# Autodesk Inventor assembly: wahacz_srodkowy_zlozenie_kopia
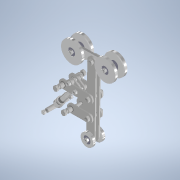
[picture p0: Inventor's stored thumbnail of the model, 180x180]
Saved by Autodesk Inventor 2020.3 (Build 243373000, 373)
## iProperties
Created: 2021-10-24
Part Number: wahacz_srodkowy_zlozenie_kopia
Document SubType Name: Assembly
Designer: patry
Author: patry
## Documents named in this file (28)
- C:\Users\patry\Desktop\Semestr 7\Inzynierka\Projekt inventor\Ariadna_inzynierka\Workspaces\Obszar roboczy\Obszar roboczy\Naped\Zawieszenie_v3\wahacz_srodkowy_zlozenie_kopia.iam
- C:\Users\patry\Desktop\Semestr 7\Inzynierka\Projekt inventor\Ariadna_inzynierka\Workspaces\Obszar roboczy\Obszar roboczy\Naped\Zawieszenie_v3\glowny_wahacz.ipt
- C:\Users\patry\Desktop\Semestr 7\Inzynierka\Projekt inventor\Ariadna_inzynierka\Workspaces\Obszar roboczy\Obszar roboczy\Naped\Zawieszenie_v3\ramie_1_wahacza.ipt
- C:\Users\patry\Desktop\Semestr 7\Inzynierka\Projekt inventor\Ariadna_inzynierka\Workspaces\Obszar roboczy\Obszar roboczy\Naped\Zawieszenie_v3\ramie_2_wahacza.ipt
- C:\Users\patry\Desktop\Semestr 7\Inzynierka\Projekt inventor\Ariadna_inzynierka\Workspaces\Obszar roboczy\Obszar roboczy\Naped\Zawieszenie_v3\tuleja_TUF106040.ipt
- C:\Users\patry\Desktop\Semestr 7\Inzynierka\Projekt inventor\Ariadna_inzynierka\Workspaces\Obszar roboczy\Obszar roboczy\Naped\Zawieszenie_v3\komplet_kol_V4.iam
- C:\Users\patry\Desktop\Semestr 7\Inzynierka\Projekt inventor\Ariadna_inzynierka\Workspaces\Obszar roboczy\Obszar roboczy\Naped\Sruby\M6_nut_5mm.ipt
- C:\Users\patry\Desktop\Semestr 7\Inzynierka\Projekt inventor\Ariadna_inzynierka\Workspaces\Obszar roboczy\Obszar roboczy\Naped\Amortyzator\Korpus.ipt
- C:\Users\patry\Desktop\Semestr 7\Inzynierka\Projekt inventor\Ariadna_inzynierka\Workspaces\Obszar roboczy\Obszar roboczy\Naped\Amortyzator\Tlok.ipt
- C:\Users\patry\Desktop\Semestr 7\Inzynierka\Projekt inventor\Ariadna_inzynierka\Workspaces\Obszar roboczy\Obszar roboczy\Naped\Amortyzator\Nakretka.ipt
- C:\Users\patry\Desktop\Semestr 7\Inzynierka\Projekt inventor\Ariadna_inzynierka\Workspaces\Obszar roboczy\Obszar roboczy\Naped\Sruby\M5_nut_5mm.ipt
- C:\Users\patry\Desktop\Semestr 7\Inzynierka\Projekt inventor\Ariadna_inzynierka\Workspaces\Obszar roboczy\Obszar roboczy\Naped\Sruby\M6_25_shaft.ipt
- C:\Users\patry\Desktop\Semestr 7\Inzynierka\Projekt inventor\Ariadna_inzynierka\Workspaces\Obszar roboczy\Obszar roboczy\Naped\Sruby\M5_70_shaft.ipt
- C:\Users\patry\Desktop\Semestr 7\Inzynierka\Projekt inventor\Ariadna_inzynierka\Workspaces\Obszar roboczy\Obszar roboczy\Naped\Sruby\M3_16_shaft.ipt
- C:\Users\patry\Desktop\Semestr 7\Inzynierka\Projekt inventor\Ariadna_inzynierka\Workspaces\Obszar roboczy\Obszar roboczy\Naped\Sruby\M3_nut_2,5mm.ipt
- C:\Users\patry\Desktop\Semestr 7\Inzynierka\Projekt inventor\Ariadna_inzynierka\Workspaces\Obszar roboczy\Obszar roboczy\Naped\Zawieszenie_v3\wspornik_amortyzatora.ipt
- C:\Users\patry\Desktop\Semestr 7\Inzynierka\Projekt inventor\Ariadna_inzynierka\Workspaces\Obszar roboczy\Obszar roboczy\Naped\Sruby\M6_40_shaft.ipt
- C:\Users\patry\Desktop\Semestr 7\Inzynierka\Projekt inventor\Ariadna_inzynierka\Workspaces\Obszar roboczy\Obszar roboczy\Naped\Sruby\tuleja_M6_M10_7.ipt
- C:\Users\patry\Desktop\Semestr 7\Inzynierka\Projekt inventor\Ariadna_inzynierka\Workspaces\Obszar roboczy\Obszar roboczy\Naped\Sruby\M6_1,25_pad.ipt
- C:\Users\patry\Desktop\Semestr 7\Inzynierka\Projekt inventor\Ariadna_inzynierka\Workspaces\Obszar roboczy\Obszar roboczy\Naped\Sruby\M6_70_shaft.ipt
- C:\Users\patry\Desktop\Semestr 7\Inzynierka\Projekt inventor\Ariadna_inzynierka\Workspaces\Obszar roboczy\Obszar roboczy\Naped\Sruby\M5_40_shaft.ipt
- M5_shaft.ipt
- C:\Users\patry\Desktop\Semestr 7\Inzynierka\Projekt inventor\Ariadna_inzynierka\Workspaces\Obszar roboczy\Obszar roboczy\Naped\Sruby\tuleja_M5_M9_20.ipt
- C:\Users\patry\Desktop\Semestr 7\Inzynierka\Projekt inventor\Ariadna_inzynierka\Workspaces\Obszar roboczy\Obszar roboczy\Naped\Sruby\tuleja_M5_M9_25.ipt
- C:\Users\patry\Desktop\Semestr 7\Inzynierka\Projekt inventor\Ariadna_inzynierka\Workspaces\Obszar roboczy\Obszar roboczy\Naped\Sruby\tuleja_M5_M9_4,5.ipt
- C:\Users\patry\Desktop\Semestr 7\Inzynierka\Projekt inventor\Ariadna_inzynierka\Workspaces\Obszar roboczy\Obszar roboczy\Naped\Kola\holder_wheel_pair.iam
- C:\Users\patry\Desktop\Semestr 7\Inzynierka\Projekt inventor\Ariadna_inzynierka\Workspaces\Obszar roboczy\Obszar roboczy\Naped\Sruby\tuleja_M6_M10_8,5.ipt
- C:\Users\patry\Desktop\Semestr 7\Inzynierka\Projekt inventor\Ariadna_inzynierka\Workspaces\Obszar roboczy\Obszar roboczy\Naped\Sruby\tuleja_M6_M10_13,5.ipt
## Components (68 placed, 26 different names)
1. glowny_wahacz:1 — Zestawiające:9, Zestawiające:12, Zestawiające:23, Zestawiające:35, Zestawiające:79, Zestawiające:106, Zestawiające:107, Zestawiające:122, Zestawiające:128, Zestawiające:136
2. ramie_1_wahacza:1 — Zestawiające:7, Zestawiające:8, Kątowe:4, Zestawiające:108, Zestawiające:109, Zestawiające:110, Równoległe:6, Zestawiające:114, Zestawiające:158, Równoległe:11, Zestawiające:159, Równoległe:12, Zestawiające:161, Zestawiające:163, Zestawiające:175, Zestawiające:179, Zestawiające:191, Zestawiające:192
3. ramie_2_wahacza:1 — Zestawiające:1, Zestawiające:2, Kątowe:1, Zestawiające:118, Zestawiające:185, Zestawiające:186
4. tuleja_TUF106040:1 — Zestawiające:1, Zestawiające:2, Kątowe:1, Zestawiające:23, Zestawiające:93
5. tuleja_TUF106040:2 — Zestawiające:184, Zestawiające:185, Zestawiające:186, Zestawiające:196
6. tuleja_TUF106040:3 — Zestawiające:190, Zestawiające:191, Zestawiające:192, Zestawiające:200
7. tuleja_TUF106040:4 — Zestawiające:7, Zestawiające:8, Kątowe:4, Zestawiające:104, Zestawiające:105, Zestawiające:111, Zestawiające:132
8. komplet_kol_V4:1 [sub-assembly] — Zestawiające:9, Zestawiające:10, Zestawiające:11, Zestawiające:12, Równoległe:13
9. glowny_wahacz:2 — Zestawiające:10, Zestawiające:11, Zestawiające:29, Zestawiające:79, Zestawiające:80, Równoległe:3, Zestawiające:82, Zestawiające:92, Zestawiające:104, Zestawiające:105, Zestawiające:124, Zestawiające:180
10. tuleja_TUF106040:5 — Zestawiające:187, Zestawiające:188, Zestawiające:189, Zestawiające:198
11. tuleja_TUF106040:6 — Zestawiające:88, Zestawiające:90, Zestawiające:106, Zestawiające:107
12. ramie_2_wahacza:2 — Równoległe:7, Zestawiające:120, Zestawiające:182, Zestawiające:183
13. tuleja_TUF106040:7 — Zestawiające:29, Zestawiające:92, Zestawiające:93, Zestawiające:112, Zestawiające:140
14. tuleja_TUF106040:8 — Zestawiające:181, Zestawiające:182, Zestawiające:183, Zestawiające:194
15. M6_nut_5mm:1 — Zestawiające:35
16. M6_nut_5mm:2 — Zestawiające:113, Zestawiające:114
17. Korpus:1 — Walcowe:1, Zestawiające:83, Równoległe:4, Zestawiające:87, Zestawiające:169, Zestawiające:171
18. Tlok:1 — Walcowe:1, Zestawiające:102, Zestawiające:103
19. Nakretka:1
20. M5_nut_5mm:1 — Zestawiające:84, Zestawiające:86, Zestawiające:87, Równoległe:9, Równoległe:10
21. M6_25_shaft:1 — Zestawiające:80, Równoległe:3, Zestawiające:81
22. M6_nut_5mm:10 — Zestawiające:81, Zestawiające:82
23. M5_70_shaft:1 — Zestawiające:83, Równoległe:4, Zestawiające:84, Zestawiające:85, Zestawiające:143, Równoległe:8, Zestawiające:168, Zestawiające:170
24. ramie_1_wahacza:3 — Zestawiające:88, Zestawiające:90, Zestawiające:116, Zestawiające:165, Zestawiające:167, Zestawiające:173, Zestawiające:177, Zestawiające:188, Zestawiające:189
25. M5_nut_5mm:2 — Zestawiające:85, Zestawiające:86
26. M3_16_shaft:1 — Zestawiające:97, Równoległe:5, Zestawiające:98, Zestawiające:100, Zestawiające:102
27. M3_nut_2,5mm:1 — Zestawiające:98, Zestawiające:99
28. M3_nut_2,5mm:2 — Zestawiające:100, Zestawiające:101
29. wspornik_amortyzatora:1 — Zestawiające:94, Zestawiające:95, Zestawiające:96, Równoległe:5, Zestawiające:99, Zestawiające:108, Zestawiające:109, Zestawiające:110
30. wspornik_amortyzatora:2 — Zestawiające:94, Zestawiające:95, Zestawiające:96, Zestawiające:97, Zestawiające:101, Zestawiające:103
31. M6_40_shaft:1 — Zestawiające:111, Równoległe:6, Zestawiające:113, Zestawiające:115, Zestawiające:121, Zestawiające:127, Zestawiające:131
32. M6_40_shaft:2 — Zestawiające:112, Równoległe:7, Zestawiające:117, Zestawiające:119, Zestawiające:123, Zestawiające:135, Zestawiające:139
33. M6_nut_5mm:11 — Zestawiające:115, Zestawiające:116
34. M6_nut_5mm:12 — Zestawiające:117, Zestawiające:118
35. M6_nut_5mm:13 — Zestawiające:119, Zestawiające:120
36. tuleja_M6_M10_7:1 — Zestawiające:121, Zestawiające:122
37. tuleja_M6_M10_7:2 — Zestawiające:123, Zestawiające:124
38. M6_1,25_pad:1 — Zestawiające:125, Zestawiające:126, Zestawiające:127, Zestawiające:128
39. M6_1,25_pad:2 — Zestawiające:125, Zestawiające:126
40. M6_1,25_pad:3 — Zestawiające:131, Zestawiające:132
41. M6_1,25_pad:4
42. M6_1,25_pad:5 — Zestawiające:135, Zestawiające:136
43. M6_1,25_pad:6
44. M6_1,25_pad:7 — Zestawiające:139, Zestawiające:140
45. M6_1,25_pad:8
46. M6_70_shaft:1 — Zestawiające:143, Zestawiające:149, Zestawiające:181, Zestawiające:184, Zestawiające:193, Zestawiające:195
47. M6_70_shaft:2 — Równoległe:8, Zestawiające:144, Zestawiające:145, Zestawiające:187, Zestawiające:190, Zestawiające:197, Zestawiające:199
48. M6_nut_5mm:14 — Zestawiające:144, Zestawiające:146
49. M6_nut_5mm:15 — Zestawiające:145, Zestawiające:146, Równoległe:9
50. M6_nut_5mm:16 — Zestawiające:148, Zestawiające:149
51. M6_nut_5mm:17 — Zestawiające:148, Równoległe:10
52. M5_shaft:1 — Zestawiające:158, Równoległe:11, Zestawiające:162, Zestawiające:164, Zestawiające:172, Zestawiające:174
53. M5_shaft:2 — Zestawiające:159, Równoległe:12, Zestawiające:160, Zestawiające:166, Zestawiające:176, Zestawiające:178
54. M5_nut_5mm:3 — Zestawiające:160, Zestawiające:161
55. M5_nut_5mm:4 — Zestawiające:162, Zestawiające:163
56. M5_nut_5mm:5 — Zestawiające:164, Zestawiające:165
57. M5_nut_5mm:6 — Zestawiające:166, Zestawiające:167
58. tuleja_M5_M9_20:1 — Zestawiające:168, Zestawiające:169
59. tuleja_M5_M9_25:1 — Zestawiające:170, Zestawiające:171
60. tuleja_M5_M9_4,5:1 — Zestawiające:172, Zestawiające:173
61. tuleja_M5_M9_4,5:2 — Zestawiające:174, Zestawiające:175
62. tuleja_M5_M9_4,5:3 — Zestawiające:176, Zestawiające:177
63. tuleja_M5_M9_4,5:4 — Zestawiające:178, Zestawiające:179
64. holder_wheel_pair:1 [sub-assembly] — Zestawiające:180, Równoległe:13
65. tuleja_M6_M10_8,5:1 — Zestawiające:193, Zestawiające:194
66. tuleja_M6_M10_13,5:1 — Zestawiające:195, Zestawiające:196
67. tuleja_M6_M10_8,5:2 — Zestawiające:199, Zestawiające:200
68. tuleja_M6_M10_13,5:2 — Zestawiające:197, Zestawiające:198
## Relationships (142: Mate 126, Flush 11, Angle 4, CylindricalJoint 1)
- Zestawiające:1 [Mate]: ramie_2_wahacza:1 ↔ tuleja_TUF106040:1
- Zestawiające:2 [Mate]: ramie_2_wahacza:1 ↔ tuleja_TUF106040:1
- Kątowe:1 [Angle] (0 deg): ramie_2_wahacza:1 ↔ tuleja_TUF106040:1
- Zestawiające:7 [Mate]: ramie_1_wahacza:1 ↔ tuleja_TUF106040:4
- Zestawiające:8 [Mate]: ramie_1_wahacza:1 ↔ tuleja_TUF106040:4
- Kątowe:4 [Angle] (0 deg): ramie_1_wahacza:1 ↔ tuleja_TUF106040:4
- Zestawiające:9 [Mate]: glowny_wahacz:1 ↔ komplet_kol_V4:1
- Zestawiające:10 [Mate]: komplet_kol_V4:1 ↔ glowny_wahacz:2
- Zestawiające:11 [Mate]: komplet_kol_V4:1 ↔ glowny_wahacz:2
- Zestawiające:12 [Mate]: glowny_wahacz:1 ↔ komplet_kol_V4:1
- Zestawiające:23 [Mate] (2.5 mm): glowny_wahacz:1 ↔ tuleja_TUF106040:1
- [Mate]: ramie_2_wahacza:2 ↔ tuleja_TUF106040:7
- [Mate]: ramie_2_wahacza:2 ↔ tuleja_TUF106040:7
- [Angle] (0 deg): ramie_2_wahacza:2 ↔ tuleja_TUF106040:7
- Zestawiające:29 [Mate] (2.5 mm): glowny_wahacz:2 ↔ tuleja_TUF106040:7
- Zestawiające:35 [Mate]: glowny_wahacz:1 ↔ M6_nut_5mm:1
- [Mate]: Korpus:1 ↔ Tlok:1
- [Angle] (0 deg): Korpus:1 ↔ Tlok:1
- [Mate]: Korpus:1 ↔ Nakretka:1
- [Mate] (5 mm): Korpus:1 ↔ Nakretka:1
- Walcowe:1 [CylindricalJoint]: Korpus:1 ↔ Tlok:1
- Zestawiające:79 [Mate]: glowny_wahacz:1 ↔ glowny_wahacz:2
- Zestawiające:80 [Mate]: glowny_wahacz:2 ↔ M6_25_shaft:1
- Równoległe:3 [Flush] (6 mm): glowny_wahacz:2 ↔ M6_25_shaft:1
- Zestawiające:81 [Mate]: M6_25_shaft:1 ↔ M6_nut_5mm:10
- Zestawiające:82 [Mate]: glowny_wahacz:2 ↔ M6_nut_5mm:10
- Zestawiające:83 [Mate]: Korpus:1 ↔ M5_70_shaft:1
- Równoległe:4 [Flush] (-30 mm): Korpus:1 ↔ M5_70_shaft:1
- Zestawiające:84 [Mate]: M5_nut_5mm:1 ↔ M5_70_shaft:1
- Zestawiające:85 [Mate]: M5_70_shaft:1 ↔ M5_nut_5mm:2
- Zestawiające:86 [Mate] (60 mm): M5_nut_5mm:1 ↔ M5_nut_5mm:2
- Zestawiające:87 [Mate] (30 mm): Korpus:1 ↔ M5_nut_5mm:1
- Zestawiające:88 [Mate]: tuleja_TUF106040:6 ↔ ramie_1_wahacza:3
- Zestawiające:90 [Mate]: tuleja_TUF106040:6 ↔ ramie_1_wahacza:3
- Zestawiające:92 [Mate]: glowny_wahacz:2 ↔ tuleja_TUF106040:7
- Zestawiające:93 [Mate]: tuleja_TUF106040:1 ↔ tuleja_TUF106040:7
- Zestawiające:94 [Mate]: wspornik_amortyzatora:1 ↔ wspornik_amortyzatora:2
- Zestawiające:95 [Mate]: wspornik_amortyzatora:1 ↔ wspornik_amortyzatora:2
- Zestawiające:96 [Mate] (5 mm): wspornik_amortyzatora:1 ↔ wspornik_amortyzatora:2
- Zestawiające:97 [Mate]: M3_16_shaft:1 ↔ wspornik_amortyzatora:2
- Równoległe:5 [Flush] (-2.5 mm): M3_16_shaft:1 ↔ wspornik_amortyzatora:1
- Zestawiające:98 [Mate]: M3_16_shaft:1 ↔ M3_nut_2,5mm:1
- Zestawiające:99 [Mate]: M3_nut_2,5mm:1 ↔ wspornik_amortyzatora:1
- Zestawiające:100 [Mate]: M3_16_shaft:1 ↔ M3_nut_2,5mm:2
- Zestawiające:101 [Mate]: M3_nut_2,5mm:2 ↔ wspornik_amortyzatora:2
- Zestawiające:102 [Mate]: Tlok:1 ↔ M3_16_shaft:1
- Zestawiające:103 [Mate]: Tlok:1 ↔ wspornik_amortyzatora:2
- Zestawiające:104 [Mate]: tuleja_TUF106040:4 ↔ glowny_wahacz:2
- Zestawiające:105 [Mate] (2.5 mm): tuleja_TUF106040:4 ↔ glowny_wahacz:2
- Zestawiające:106 [Mate] (2.5 mm): glowny_wahacz:1 ↔ tuleja_TUF106040:6
- Zestawiające:107 [Mate]: glowny_wahacz:1 ↔ tuleja_TUF106040:6
- Zestawiające:108 [Mate]: ramie_1_wahacza:1 ↔ wspornik_amortyzatora:1
- Zestawiające:109 [Mate]: ramie_1_wahacza:1 ↔ wspornik_amortyzatora:1
- Zestawiające:110 [Mate] (4.5 mm): ramie_1_wahacza:1 ↔ wspornik_amortyzatora:1
- Zestawiające:111 [Mate]: tuleja_TUF106040:4 ↔ M6_40_shaft:1
- Równoległe:6 [Flush] (7 mm): ramie_1_wahacza:1 ↔ M6_40_shaft:1
- Zestawiające:112 [Mate]: tuleja_TUF106040:7 ↔ M6_40_shaft:2
- Równoległe:7 [Flush] (7 mm): ramie_2_wahacza:2 ↔ M6_40_shaft:2
- Zestawiające:113 [Mate]: M6_nut_5mm:2 ↔ M6_40_shaft:1
- Zestawiające:114 [Mate]: ramie_1_wahacza:1 ↔ M6_nut_5mm:2
- Zestawiające:115 [Mate]: M6_40_shaft:1 ↔ M6_nut_5mm:11
- Zestawiające:116 [Mate]: ramie_1_wahacza:3 ↔ M6_nut_5mm:11
- Zestawiające:117 [Mate]: M6_40_shaft:2 ↔ M6_nut_5mm:12
- Zestawiające:118 [Mate]: ramie_2_wahacza:1 ↔ M6_nut_5mm:12
- Zestawiające:119 [Mate]: M6_40_shaft:2 ↔ M6_nut_5mm:13
- Zestawiające:120 [Mate]: ramie_2_wahacza:2 ↔ M6_nut_5mm:13
- Zestawiające:121 [Mate]: M6_40_shaft:1 ↔ tuleja_M6_M10_7:1
- Zestawiające:122 [Mate]: glowny_wahacz:1 ↔ tuleja_M6_M10_7:1
- Zestawiające:123 [Mate]: M6_40_shaft:2 ↔ tuleja_M6_M10_7:2
- Zestawiające:124 [Mate]: glowny_wahacz:2 ↔ tuleja_M6_M10_7:2
- Zestawiające:125 [Mate]: M6_1,25_pad:1 ↔ M6_1,25_pad:2
- Zestawiające:126 [Mate]: M6_1,25_pad:1 ↔ M6_1,25_pad:2
- Zestawiające:127 [Mate]: M6_40_shaft:1 ↔ M6_1,25_pad:1
- Zestawiające:128 [Mate]: glowny_wahacz:1 ↔ M6_1,25_pad:1
- [Mate]: M6_1,25_pad:3 ↔ M6_1,25_pad:4
- [Mate]: M6_1,25_pad:3 ↔ M6_1,25_pad:4
- Zestawiające:131 [Mate]: M6_40_shaft:1 ↔ M6_1,25_pad:3
- Zestawiające:132 [Mate]: tuleja_TUF106040:4 ↔ M6_1,25_pad:3
- [Mate]: M6_1,25_pad:5 ↔ M6_1,25_pad:6
- [Mate]: M6_1,25_pad:5 ↔ M6_1,25_pad:6
- Zestawiające:135 [Mate]: M6_40_shaft:2 ↔ M6_1,25_pad:5
- Zestawiające:136 [Mate]: glowny_wahacz:1 ↔ M6_1,25_pad:5
- [Mate]: M6_1,25_pad:7 ↔ M6_1,25_pad:8
- [Mate]: M6_1,25_pad:7 ↔ M6_1,25_pad:8
- Zestawiające:139 [Mate]: M6_40_shaft:2 ↔ M6_1,25_pad:7
- Zestawiające:140 [Mate]: tuleja_TUF106040:7 ↔ M6_1,25_pad:7
- Zestawiające:143 [Mate]: M5_70_shaft:1 ↔ M6_70_shaft:1
- Równoległe:8 [Flush]: M5_70_shaft:1 ↔ M6_70_shaft:2
- Zestawiające:144 [Mate]: M6_70_shaft:2 ↔ M6_nut_5mm:14
- Zestawiające:145 [Mate]: M6_70_shaft:2 ↔ M6_nut_5mm:15
- Zestawiające:146 [Mate] (60 mm): M6_nut_5mm:14 ↔ M6_nut_5mm:15
- Równoległe:9 [Flush]: M5_nut_5mm:1 ↔ M6_nut_5mm:15
- [Mate] (60 mm): M6_nut_5mm:16 ↔ M6_nut_5mm:17
- Zestawiające:148 [Mate]: M6_nut_5mm:16 ↔ M6_nut_5mm:17
- Zestawiające:149 [Mate]: M6_70_shaft:1 ↔ M6_nut_5mm:16
- Równoległe:10 [Flush]: M5_nut_5mm:1 ↔ M6_nut_5mm:17
- Zestawiające:158 [Mate]: ramie_1_wahacza:1 ↔ M5_shaft:1
- Równoległe:11 [Flush] (7 mm): ramie_1_wahacza:1 ↔ M5_shaft:1
- Zestawiające:159 [Mate]: ramie_1_wahacza:1 ↔ M5_shaft:2
- Równoległe:12 [Flush] (7 mm): ramie_1_wahacza:1 ↔ M5_shaft:2
- Zestawiające:160 [Mate]: M5_shaft:2 ↔ M5_nut_5mm:3
- Zestawiające:161 [Mate]: ramie_1_wahacza:1 ↔ M5_nut_5mm:3
- Zestawiające:162 [Mate]: M5_shaft:1 ↔ M5_nut_5mm:4
- Zestawiające:163 [Mate]: ramie_1_wahacza:1 ↔ M5_nut_5mm:4
- Zestawiające:164 [Mate]: M5_shaft:1 ↔ M5_nut_5mm:5
- Zestawiające:165 [Mate]: ramie_1_wahacza:3 ↔ M5_nut_5mm:5
- Zestawiające:166 [Mate]: M5_shaft:2 ↔ M5_nut_5mm:6
- Zestawiające:167 [Mate]: ramie_1_wahacza:3 ↔ M5_nut_5mm:6
- Zestawiające:168 [Mate]: M5_70_shaft:1 ↔ tuleja_M5_M9_20:1
- Zestawiające:169 [Mate]: Korpus:1 ↔ tuleja_M5_M9_20:1
- Zestawiające:170 [Mate]: M5_70_shaft:1 ↔ tuleja_M5_M9_25:1
- Zestawiające:171 [Mate]: Korpus:1 ↔ tuleja_M5_M9_25:1
- Zestawiające:172 [Mate]: M5_shaft:1 ↔ tuleja_M5_M9_4,5:1
- Zestawiające:173 [Mate]: ramie_1_wahacza:3 ↔ tuleja_M5_M9_4,5:1
- Zestawiające:174 [Mate]: M5_shaft:1 ↔ tuleja_M5_M9_4,5:2
- Zestawiające:175 [Mate]: ramie_1_wahacza:1 ↔ tuleja_M5_M9_4,5:2
- Zestawiające:176 [Mate]: M5_shaft:2 ↔ tuleja_M5_M9_4,5:3
- Zestawiające:177 [Mate]: ramie_1_wahacza:3 ↔ tuleja_M5_M9_4,5:3
- Zestawiające:178 [Mate]: M5_shaft:2 ↔ tuleja_M5_M9_4,5:4
- Zestawiające:179 [Mate]: ramie_1_wahacza:1 ↔ tuleja_M5_M9_4,5:4
- Zestawiające:180 [Mate]: glowny_wahacz:2 ↔ holder_wheel_pair:1
- Równoległe:13 [Flush]: komplet_kol_V4:1 ↔ holder_wheel_pair:1
- Zestawiające:181 [Mate]: tuleja_TUF106040:8 ↔ M6_70_shaft:1
- Zestawiające:182 [Mate]: ramie_2_wahacza:2 ↔ tuleja_TUF106040:8
- Zestawiające:183 [Mate]: ramie_2_wahacza:2 ↔ tuleja_TUF106040:8
- Zestawiające:184 [Mate]: tuleja_TUF106040:2 ↔ M6_70_shaft:1
- Zestawiające:185 [Mate]: ramie_2_wahacza:1 ↔ tuleja_TUF106040:2
- Zestawiające:186 [Mate]: ramie_2_wahacza:1 ↔ tuleja_TUF106040:2
- Zestawiające:187 [Mate]: tuleja_TUF106040:5 ↔ M6_70_shaft:2
- Zestawiające:188 [Mate]: tuleja_TUF106040:5 ↔ ramie_1_wahacza:3
- Zestawiające:189 [Mate]: tuleja_TUF106040:5 ↔ ramie_1_wahacza:3
- Zestawiające:190 [Mate]: tuleja_TUF106040:3 ↔ M6_70_shaft:2
- Zestawiające:191 [Mate]: ramie_1_wahacza:1 ↔ tuleja_TUF106040:3
- Zestawiające:192 [Mate]: ramie_1_wahacza:1 ↔ tuleja_TUF106040:3
- Zestawiające:193 [Mate]: M6_70_shaft:1 ↔ tuleja_M6_M10_8,5:1
- Zestawiające:194 [Mate]: tuleja_TUF106040:8 ↔ tuleja_M6_M10_8,5:1
- Zestawiające:195 [Mate]: M6_70_shaft:1 ↔ tuleja_M6_M10_13,5:1
- Zestawiające:196 [Mate]: tuleja_TUF106040:2 ↔ tuleja_M6_M10_13,5:1
- Zestawiające:197 [Mate]: M6_70_shaft:2 ↔ tuleja_M6_M10_13,5:2
- Zestawiające:198 [Mate]: tuleja_TUF106040:5 ↔ tuleja_M6_M10_13,5:2
- Zestawiające:199 [Mate]: M6_70_shaft:2 ↔ tuleja_M6_M10_8,5:2
- Zestawiające:200 [Mate]: tuleja_TUF106040:3 ↔ tuleja_M6_M10_8,5:2
## Named parameters: d41_d4 = 0 deg, d43_d0 = 0 mm, d44_d1 = 0 mm, d83_d6 = -2 mm, d84_d7 = -2 mm, d85_d8 = -13 mm, d86_d0 = 0 mm, d87_d1 = 0 deg, d88_d3 = 0 mm, d89_d4 = 5 mm, d90_d5 = 0 deg, d158_d154 = 0 mm, d159_d155 = 0 mm, d162_d154 = 0 mm, d163_d155 = 0 mm, d166_d154 = 0 mm, d167_d155 = 0 mm, d178_d176 = 60 mm
